# Autodesk Inventor assembly: ASM_Micron_OCT_Int
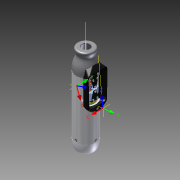
[picture p0: Inventor's stored thumbnail of the model, 180x180]
Saved by Autodesk Inventor 2011 SP2 (Build 150309200, 309)
## iProperties
Created: 2011-10-07
Part Number: ASM_Micron_OCT_Int
Document SubType Name: Assembly
Designer: sungwook
Author: sungwook
## Documents named in this file (14)
- C:\Users\sungwook\Documents\Inventor\Micron20_Base_Tube_Adjst\Assembly\OCT\ASM_Micron_OCT_Integration.iam
- C:\Users\sungwook\Documents\Inventor\Micron20_Base_Tube_Adjst\Assembly\OCT\ASM_Micron_OCT_Probe.iam
- C:\Users\sungwook\Documents\Inventor\Micron20_Base_Tube_Adjst\Parts\ASAP\Handle_ASAP.iam
- C:\Users\sungwook\Documents\Inventor\Micron20_Base_Tube_Adjst\Parts\Electronics\PCB_Stack.iam
- C:\Users\sungwook\Documents\Inventor\Micron20_Base_Tube_Adjst\06082012_Outer_Tube\Outer_Tube.ipt
- C:\Users\sungwook\Documents\Inventor\Content Center Files\R2011\en-US\ANSI B18.6.3(00)\ANSI B18.6.3 - 0-80 UNF - 0.1875(32).ipt
- C:\Users\sungwook\Documents\Inventor\Micron20_Base_Tube_Adjst\Parts\Handle\Ver2(Al_RP)\Handle_2_Back_rev2.ipt
- C:\Users\sungwook\Documents\Inventor\Micron20_Base_Tube_Adjst\04192012_New_Front_2pcs\New_Front_Base_rev.ipt
- C:\Users\sungwook\Documents\Inventor\Micron20_Base_Tube_Adjst\04192012_New_Front_2pcs\New_Front_Upper_rev.ipt
- C:\Users\sungwook\Documents\Inventor\Micron20_Base_Tube_Adjst\04192012_New_Front_2pcs\New_Front_Upper_rev_v2.ipt
- C:\Users\sungwook\Documents\Inventor\Micron20_Base_Tube_Adjst\04192012_New_Front_2pcs\New_Front_Upper_rev_v3.ipt
- C:\Users\sungwook\Documents\Inventor\Content Center Files\R2011\en-US\ANSI B18.6.3(00)\ANSI B18.6.3 - 2-56 UNC - 0.1875(32).ipt
- C:\Users\sungwook\Documents\Inventor\Content Center Files\R2011\en-US\ANSI B18.6.3(00)\ANSI B18.6.3 - 2-56 UNC - 0.125(32).ipt
- C:\Users\sungwook\Documents\Inventor\Micron20_Base_Tube_Adjst\Parts\Main\Guide_Tube_Base.ipt
## Components (16 placed, 13 different names)
1. (0,0,0) [sub-assembly] — Mate:2, Mate:55, Mate:73, Mate:74, Mate:107, Mate:108, Mate:125
2. Handle_ASAP:1 [sub-assembly] — Mate:55
3. PCB_Stack:1 [sub-assembly] — Flush:73, Mate:73, Mate:74, Mate:125
4. Handle_2_Back_rev2:1 — Mate:109, Mate:110, Mate:111, Mate:123, Mate:124, Mate:126, Flush:125
5. Outer_Tube:1 — Mate:104, Mate:105, Mate:108, Mate:109, Mate:111, Mate:114, Mate:117, Mate:118, Mate:119, Flush:122, Flush:124
6. New_Front_Base_rev:1 — Mate:112, Mate:113, Mate:114, Flush:74, Mate:120, Flush:121, Mate:121, Flush:123
7. New_Front_Upper_rev:1 — Mate:117, Flush:74, Mate:118, Mate:119
8. New_Front_Upper_rev_v2:1 — Mate:120, Flush:121, Flush:122, Mate:122
9. New_Front_Upper_rev_v3:1 — Mate:121, Flush:123, Flush:124
10. Cross Recessed 100° Flat Countersunk Head Machine Screw - Type I - Inch 2-56 UNC x 0.1875:1 — Mate:122
11. Cross Recessed 100° Flat Countersunk Head Machine Screw - Type I - Inch 2-56 UNC x 0.125:1 — Mate:123
12. Cross Recessed 100° Flat Countersunk Head Machine Screw - Type I - Inch 2-56 UNC x 0.125:2 — Mate:124
13. Guide_Tube_Base:1 — Mate:126, Flush:125
14. Cross Recessed 100° Flat Countersunk Head Machine Screw - Type I - Inch 0-80 UNF x 0.1875:1 — Mate:107
15. Cross Recessed 100° Flat Countersunk Head Machine Screw - Type I - Inch 0-80 UNF x 0.1875:2
16. Cross Recessed 100° Flat Countersunk Head Machine Screw - Type I - Inch 0-80 UNF x 0.1875:3
## Component patterns: (3 elements, first: Cross Recessed 100° Flat Countersunk Head Machine Screw - Type I - Inch 0-80 UNF x 0.1875:1)
## Relationships (31: Mate 24, Flush 7)
- Mate:2: (0,0,0)
- Mate:55: (0,0,0) ↔ Handle_ASAP:1
- Flush:73: PCB_Stack:1
- Mate:73: (0,0,0) ↔ PCB_Stack:1
- Mate:74: (0,0,0) ↔ PCB_Stack:1
- Mate:104: Outer_Tube:1
- Mate:105: Outer_Tube:1
- Mate:108: (0,0,0) ↔ Outer_Tube:1
- Mate:109: Handle_2_Back_rev2:1 ↔ Outer_Tube:1
- Mate:110: Handle_2_Back_rev2:1
- Mate:111: Handle_2_Back_rev2:1 ↔ Outer_Tube:1
- Mate:112: New_Front_Base_rev:1
- Mate:113: New_Front_Base_rev:1
- Mate:114: Outer_Tube:1 ↔ New_Front_Base_rev:1
- Mate:117: Outer_Tube:1 ↔ New_Front_Upper_rev:1
- Flush:74: New_Front_Base_rev:1 ↔ New_Front_Upper_rev:1
- Mate:118: Outer_Tube:1 ↔ New_Front_Upper_rev:1
- Mate:119: Outer_Tube:1 ↔ New_Front_Upper_rev:1
- Mate:120: New_Front_Base_rev:1 ↔ New_Front_Upper_rev_v2:1
- Flush:121: New_Front_Base_rev:1 ↔ New_Front_Upper_rev_v2:1
- Flush:122: Outer_Tube:1 ↔ New_Front_Upper_rev_v2:1
- Mate:121: New_Front_Base_rev:1 ↔ New_Front_Upper_rev_v3:1
- Flush:123: New_Front_Base_rev:1 ↔ New_Front_Upper_rev_v3:1
- Flush:124: Outer_Tube:1 ↔ New_Front_Upper_rev_v3:1
- Mate:125: (0,0,0) ↔ PCB_Stack:1
- Mate:126: Handle_2_Back_rev2:1 ↔ Guide_Tube_Base:1
- Flush:125 (5 mm): Handle_2_Back_rev2:1 ↔ Guide_Tube_Base:1
- Mate:107: (0,0,0) ↔ Cross Recessed 100° Flat Countersunk Head Machine Screw - Type I - Inch 0-80 UNF x 0.1875:1
- Mate:122: New_Front_Upper_rev_v2:1 ↔ Cross Recessed 100° Flat Countersunk Head Machine Screw - Type I - Inch 2-56 UNC x 0.1875:1
- Mate:123: Handle_2_Back_rev2:1 ↔ Cross Recessed 100° Flat Countersunk Head Machine Screw - Type I - Inch 2-56 UNC x 0.125:1
- Mate:124: Handle_2_Back_rev2:1 ↔ Cross Recessed 100° Flat Countersunk Head Machine Screw - Type I - Inch 2-56 UNC x 0.125:2
